# Autodesk Inventor assembly: ГОРИЗОНТАЛЬНЫЙ ЗАХВАТ
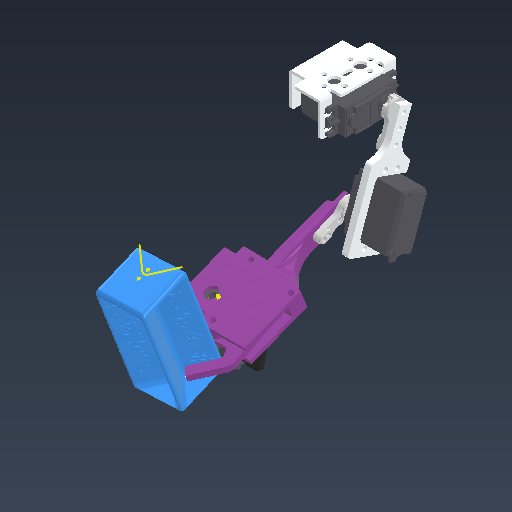
[picture p0: Inventor's stored thumbnail of the model, 512x512]
Saved by Autodesk Inventor 2025 (Build 290162000, 162)
## iProperties
Created: 2025-01-28
Part Number: ГОРИЗОНТАЛЬНЫЙ ЗАХВАТ
Document SubType Name: Assembly
Designer: GameHD
Author: GameHD
## Documents named in this file (8)
- C:\Users\GameHD\Desktop\phantom 16950\ГОРИЗОНТАЛЬНЫЙ ЗАХВАТ.iam
- C:\Users\GameHD\Desktop\phantom 16950\39060_txm-standard servo bracket\39060_txm-standard servo bracket_MIR1.ipt
- C:\Users\GameHD\Desktop\phantom 16950\2000-0025-0002\2000-0025-0002_MIR2.ipt
- C:\Users\GameHD\Desktop\phantom 16950\DS3225_MG_metal_horn\DS3225_MG_metal_horn_MIR1.ipt
- C:\Users\GameHD\Desktop\phantom 16950\2000-0025-0002\2000-0025-0002_MIR2_MIR1.ipt
- C:\Users\GameHD\Desktop\phantom 16950\DS3225_MG_metal_horn\DS3225_MG_metal_horn_MIR1_MIR.ipt
- C:\Users\GameHD\Desktop\phantom 16950\держать писюны 3ч_MIR.ipt
- C:\Users\GameHD\Desktop\phantom 16950\писюны_MIR2_MIR.iam
## Components (7 placed, 7 different names)
1. 39060_txm-standard servo bracket_MIR1:1
2. 2000-0025-0002_MIR2:1
3. DS3225_MG_metal_horn_MIR1:1
4. 2000-0025-0002_MIR2_MIR1:1
5. DS3225_MG_metal_horn_MIR1_MIR:1
6. держать писюны 3ч_MIR:1
7. писюны_MIR2_MIR:1 [sub-assembly]
## Relationships (15: Mate 12, Flush 3)
- [Mate]: 39060_txm-standard servo bracket_MIR1:1 ↔ 2000-0025-0002_MIR2:1
- [Mate] (1 mm): 2000-0025-0002_MIR2:1 ↔ DS3225_MG_metal_horn_MIR1:1
- [Mate]: 2000-0025-0002_MIR2:1 ↔ DS3225_MG_metal_horn_MIR1:1
- [Mate]: 2000-0025-0002_MIR2_MIR1:1 ↔ DS3225_MG_metal_horn_MIR1_MIR:1
- [Mate] (1 mm): 2000-0025-0002_MIR2_MIR1:1 ↔ DS3225_MG_metal_horn_MIR1_MIR:1
- [Mate]: 2000-0025-0002_MIR2_MIR1:1 ↔ держать писюны 3ч_MIR:1
- [Mate]: 2000-0025-0002_MIR2_MIR1:1 ↔ держать писюны 3ч_MIR:1
- [Mate] (1 mm): 2000-0025-0002_MIR2_MIR1:1 ↔ держать писюны 3ч_MIR:1
- [Flush] (-1 mm): DS3225_MG_metal_horn_MIR1:1 ↔ держать писюны 3ч_MIR:1
- [Mate] (2 mm): DS3225_MG_metal_horn_MIR1:1 ↔ держать писюны 3ч_MIR:1
- [Mate]: DS3225_MG_metal_horn_MIR1:1 ↔ держать писюны 3ч_MIR:1
- [Flush] (-0.5 mm): DS3225_MG_metal_horn_MIR1_MIR:1 ↔ писюны_MIR2_MIR:1
- [Mate]: DS3225_MG_metal_horn_MIR1_MIR:1 ↔ писюны_MIR2_MIR:1
- [Mate] (4.5 mm): 39060_txm-standard servo bracket_MIR1:1 ↔ 2000-0025-0002_MIR2:1
- [Flush] (2 mm): 39060_txm-standard servo bracket_MIR1:1 ↔ 2000-0025-0002_MIR2:1
